# Autodesk Inventor assembly: 203
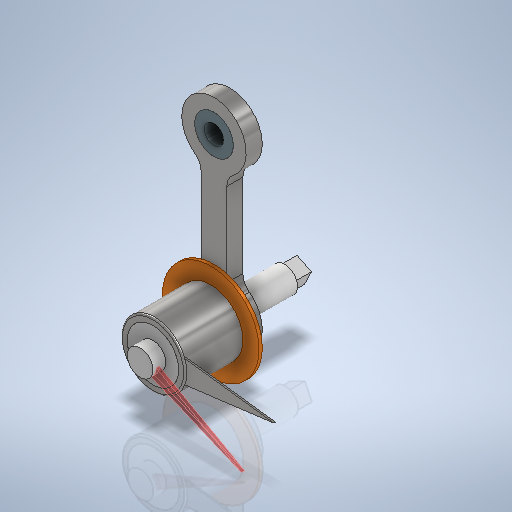
[picture p0: Inventor's stored thumbnail of the model, 512x512]
Saved by Autodesk Inventor 2025.1 (Build 291241000, 241)
## iProperties
Created: 2024-09-02
Part Number: 203
Document SubType Name: Assembly
Designer: ffogue
Author: ffogue
## Documents named in this file (6)
- C:\Users\ffogue\Documents\Inventor\Planetary Gear\203.iam
- C:\Users\ffogue\Documents\Inventor\Planetary Gear\203 part 1.ipt
- C:\Users\ffogue\Documents\Inventor\Planetary Gear\Sicherung.ipt
- C:\Users\ffogue\Documents\Inventor\Planetary Gear\203 part 3.ipt
- C:\Users\ffogue\Documents\Inventor\Planetary Gear\204 part 1.ipt
- C:\Users\ffogue\Documents\Inventor\Planetary Gear\202 part 3.ipt
## Components (5 placed, 5 different names)
1. 203 part 1:1 — Insert:1, Mate:1, Flush:1, Mate:2, Flush:2, Mate:8, Flush:4, Angle:2
2. Sicherung:1 — Insert:1
3. 203 part 3:1 — Mate:1, Flush:1
4. 204 part 1:1 — Mate:2, Flush:2
5. 202 part 3:1 — Mate:8, Flush:4, Angle:2
## Relationships (8: Mate 3, Flush 3, Insert 1, Angle 1)
- Insert:1 (-1 mm): 203 part 1:1 ↔ Sicherung:1
- Mate:1: 203 part 1:1 ↔ 203 part 3:1
- Flush:1: 203 part 1:1 ↔ 203 part 3:1
- Mate:2: 203 part 1:1 ↔ 204 part 1:1
- Flush:2: 203 part 1:1 ↔ 204 part 1:1
- Mate:8: 203 part 1:1 ↔ 202 part 3:1
- Flush:4 (-3.5 mm): 203 part 1:1 ↔ 202 part 3:1
- Angle:2 (30 deg): 203 part 1:1 ↔ 202 part 3:1
